# Autodesk Inventor assembly: фуллл
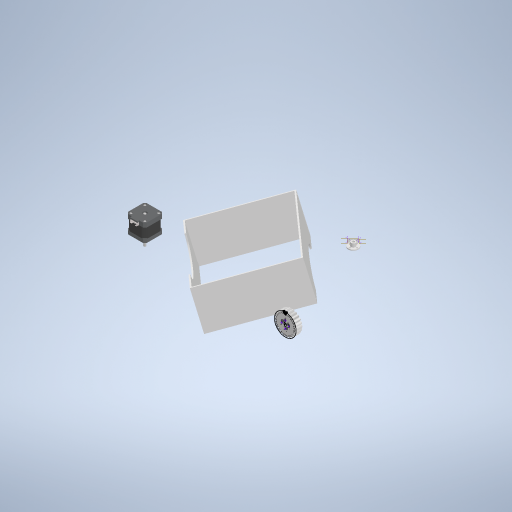
[picture p0: Inventor's stored thumbnail of the model, 512x512]
Saved by Autodesk Inventor 2024.2 (Build 282272000, 272)
## iProperties
Created: 2025-11-20
Part Number: фуллл
Document SubType Name: Assembly
Designer: Zakhar
Author: Zakhar
## Documents named in this file (6)
- C:\Users\Zakhar\Documents\Деталь ВсОШ\фуллл.iam
- C:\Users\Zakhar\Documents\Деталь ВсОШ\NEMA17 42-40.ipt
- C:\Users\Zakhar\Documents\Деталь ВсОШ\боковая стенка.ipt
- C:\Users\Zakhar\Documents\Деталь ВсОШ\Муфта.ipt
- C:\Users\Zakhar\Documents\Деталь ВсОШ\передняя стенка.ipt
- C:\Users\Zakhar\Documents\Деталь ВсОШ\Шест.ipt
## Components (7 placed, 5 different names)
1. NEMA17 42-40:1
2. боковая стенка:1 — Жесткий:1
3. Муфта:1
4. передняя стенка:1 — Жесткий:1
5. Шест:1
6. боковая стенка:2 — Жесткий:2
7. передняя стенка:2 — Жесткий:2
## Relationships (2: WeldJoint 2)
- Жесткий:1 [WeldJoint]: боковая стенка:1 ↔ передняя стенка:1
- Жесткий:2 [WeldJoint]: боковая стенка:2 ↔ передняя стенка:2
